# Autodesk Inventor assembly: 20X20 lift
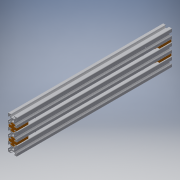
[picture p0: Inventor's stored thumbnail of the model, 180x180]
Saved by Autodesk Inventor 2019 (Build 230136000, 136)
## iProperties
Created: 2018-10-27
Part Number: 20X20 lift
Document SubType Name: Assembly
Designer: User
Author: User
## Documents named in this file (3)
- C:\Robotics\CAD\2018-19_CAD\Collection\20X20 lift.iam
- C:\Robotics\CAD\2018-19_CAD\Collection\20X20 lift conecter.ipt
- C:\Robotics\CAD\COTSParts\Bosch Extrusion\Bosch 20x20 13 in - Real.ipt
## Components (7 placed, 2 different names)
1. 20X20 lift conecter:2 — Flush:1, Mate:1, Mate:2, Mate:9
2. 20X20 lift conecter:5 — Mate:3, Mate:7, Flush:11, Mate:9
3. Bosch 20x20 13 in - Real:1 — Flush:1, Mate:1, Mate:2, Mate:3, Flush:7
4. Bosch 20x20 13 in - Real:3 — Mate:8, Flush:9, Flush:10
5. 20X20 lift conecter:6 — Mate:10
6. 20X20 lift conecter:7 — Mate:8, Flush:10, Mate:10
7. Bosch 20x20 13 in - Real:4 — Mate:7, Flush:7, Flush:9, Flush:11
## Relationships (17: Mate 10, Flush 7)
- Flush:1: 20X20 lift conecter:2 ↔ Bosch 20x20 13 in - Real:1
- Mate:1 (0.4572 mm): 20X20 lift conecter:2 ↔ Bosch 20x20 13 in - Real:1
- Mate:2 (1.524 mm): 20X20 lift conecter:2 ↔ Bosch 20x20 13 in - Real:1
- Mate:3 (0.4572 mm): 20X20 lift conecter:5 ↔ Bosch 20x20 13 in - Real:1
- [Flush]: 20X20 lift conecter:6 ↔ Bosch 20x20 13 in - Real:4
- [Mate] (0.4572 mm): 20X20 lift conecter:6 ↔ Bosch 20x20 13 in - Real:4
- [Mate] (1.524 mm): 20X20 lift conecter:6 ↔ Bosch 20x20 13 in - Real:4
- [Mate] (0.4572 mm): 20X20 lift conecter:7 ↔ Bosch 20x20 13 in - Real:4
- [Flush]: 20X20 lift conecter:6 ↔ 20X20 lift conecter:7
- Mate:7 (0.4572 mm): 20X20 lift conecter:5 ↔ Bosch 20x20 13 in - Real:4
- Flush:7: Bosch 20x20 13 in - Real:1 ↔ Bosch 20x20 13 in - Real:4
- Mate:8 (0.4572 mm): Bosch 20x20 13 in - Real:3 ↔ 20X20 lift conecter:7
- Flush:9: Bosch 20x20 13 in - Real:3 ↔ Bosch 20x20 13 in - Real:4
- Flush:10: Bosch 20x20 13 in - Real:3 ↔ 20X20 lift conecter:7
- Flush:11: 20X20 lift conecter:5 ↔ Bosch 20x20 13 in - Real:4
- Mate:9: 20X20 lift conecter:2 ↔ 20X20 lift conecter:5
- Mate:10: 20X20 lift conecter:6 ↔ 20X20 lift conecter:7
## Named parameters: d6_d2 = 1.524 mm, d8_d4 = 0.4572 mm, d9_d5 = 0 mm, d10_d0 = 0 mm, d11_d1 = 0.4572 mm
